# Autodesk Inventor assembly: scaled-case
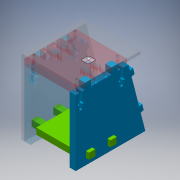
[picture p0: Inventor's stored thumbnail of the model, 180x180]
Saved by Autodesk Inventor 2017 (Build 210142000, 142)
## iProperties
Created: 2017-02-28
Part Number: scaled-case
Document SubType Name: Assembly
Designer: John
Author: John
## Documents named in this file (6)
- C:\Users\John\Dropbox\ECE115\pinball-project\scaled-case.iam
- C:\Users\John\Dropbox\ECE115\pinball-project\wall-front-scale.ipt
- C:\Users\John\Dropbox\ECE115\pinball-project\pinball-case-left-wal-scaledl.ipt
- C:\Users\John\Dropbox\ECE115\pinball-project\pinball-case-left-wall-outer-scaled.ipt
- C:\Users\John\Dropbox\ECE115\pinball-project\wall-front-outer-scaled.ipt
- C:\Users\John\Dropbox\ECE115\pinball-project\wall-back-scaled.ipt
## Components (6 placed, 5 different names)
1. wall-front-scale:1 — Mate:3, Flush:2, Flush:3, Flush:4, Flush:5, Flush:10, Flush:11, Mate:9, Flush:12, Mate:10
2. pinball-case-left-wal-scaledl:1 — Flush:10, Flush:11, Mate:9, Flush:12, Mate:11
3. pinball-case-left-wal-scaledl:2 — Mate:3, Flush:2, Flush:3
4. pinball-case-left-wall-outer-scaled:1 — Flush:4, Flush:5, Flush:9, Mate:7, Mate:8, Flush:13, Mate:11, Flush:14
5. wall-front-outer-scaled:1 — Mate:10, Flush:13, Flush:14
6. wall-back-scaled:1 — Flush:9, Mate:7, Mate:8
## Relationships (16: Flush 10, Mate 6)
- Mate:3: wall-front-scale:1 ↔ pinball-case-left-wal-scaledl:2
- Flush:2: wall-front-scale:1 ↔ pinball-case-left-wal-scaledl:2
- Flush:3: wall-front-scale:1 ↔ pinball-case-left-wal-scaledl:2
- Flush:4: wall-front-scale:1 ↔ pinball-case-left-wall-outer-scaled:1
- Flush:5: wall-front-scale:1 ↔ pinball-case-left-wall-outer-scaled:1
- Flush:9: pinball-case-left-wall-outer-scaled:1 ↔ wall-back-scaled:1
- Mate:7: pinball-case-left-wall-outer-scaled:1 ↔ wall-back-scaled:1
- Mate:8: pinball-case-left-wall-outer-scaled:1 ↔ wall-back-scaled:1
- Flush:10: wall-front-scale:1 ↔ pinball-case-left-wal-scaledl:1
- Flush:11: wall-front-scale:1 ↔ pinball-case-left-wal-scaledl:1
- Mate:9: wall-front-scale:1 ↔ pinball-case-left-wal-scaledl:1
- Flush:12: wall-front-scale:1 ↔ pinball-case-left-wal-scaledl:1
- Mate:10: wall-front-scale:1 ↔ wall-front-outer-scaled:1
- Flush:13: pinball-case-left-wall-outer-scaled:1 ↔ wall-front-outer-scaled:1
- Mate:11: pinball-case-left-wal-scaledl:1 ↔ pinball-case-left-wall-outer-scaled:1
- Flush:14: pinball-case-left-wall-outer-scaled:1 ↔ wall-front-outer-scaled:1
